# Autodesk Inventor assembly: Truss
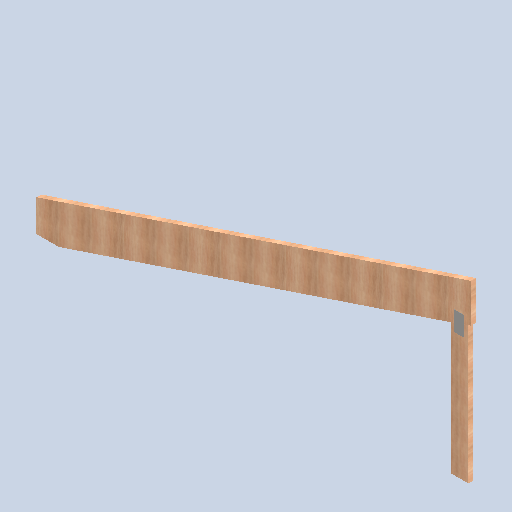
[picture p0: Inventor's stored thumbnail of the model, 512x512]
Saved by Autodesk Inventor 2025 (Build 290162010, 162A)
## iProperties
Created: 2024-09-16
Part Number: Truss
Document SubType Name: Assembly
Designer: Tom
Author: Tom
## Documents named in this file (4)
- C:\Users\Tom\Documents\Inventor\Mobility\Additional_Building\Truss.iam
- C:\Users\Tom\Documents\Inventor\Mobility\Additional_Building\Rafter.ipt
- C:\Users\Tom\Documents\Inventor\Mobility\Additional_Building\Stud_With_Height_42.1875_Inches.ipt
- C:\Users\Tom\Documents\Inventor\Mobility\Additional_Building\Mending_Plate.ipt
## Components (4 placed, 3 different names)
1. Rafter:1 — Flush:2, Mate:1, Mate:2, Flush:3, Mate:3, Mate:4, Flush:5
2. Stud_With_Height_42.1875_Inches:1 — Flush:1, Mate:1, Flush:4, Flush:5, Flush:6
3. Mending_Plate:1 — Mate:2, Flush:3, Flush:4
4. Mending_Plate:2 — Mate:3, Mate:4, Flush:6
## Relationships (10: Flush 6, Mate 4)
- Flush:1: Stud_With_Height_42.1875_Inches:1
- Flush:2: Rafter:1
- Mate:1: Rafter:1 ↔ Stud_With_Height_42.1875_Inches:1
- Mate:2: Rafter:1 ↔ Mending_Plate:1
- Flush:3 (-101.6 mm): Rafter:1 ↔ Mending_Plate:1
- Flush:4 (31.75 mm): Stud_With_Height_42.1875_Inches:1 ↔ Mending_Plate:1
- Mate:3: Rafter:1 ↔ Mending_Plate:2
- Mate:4 (-50.8 mm): Rafter:1 ↔ Mending_Plate:2
- Flush:5: Rafter:1 ↔ Stud_With_Height_42.1875_Inches:1
- Flush:6 (31.75 mm): Stud_With_Height_42.1875_Inches:1 ↔ Mending_Plate:2
